# Autodesk Inventor assembly: SG90 - Micro Servo 9g - Tower Pro
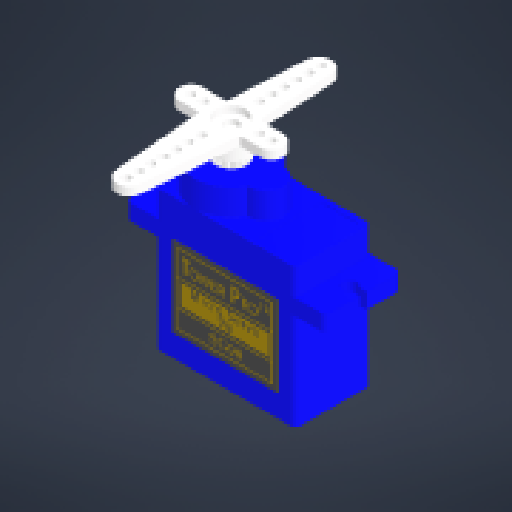
[picture p0: Inventor's stored thumbnail of the model, 512x512]
Saved by Autodesk Inventor 2024 (Build 280153000, 153)
## iProperties
Created: 2019-03-11
Part Number: SG90 - Micro Servo 9g - Tower Pro
Description: STEP AP214
Document SubType Name: Assembly
Designer: Daniel
Sending System: SolidWorks 2018
Preprocessor: SwSTEP 2.0
Title: SG90 - Micro Servo 9g - Tower Pro.STEP
Revision Number: ANY
## Documents named in this file (3)
- C:\Users\Daniel\Desktop\pmik_2024l_jd\mechanical\STEPS\SG90 - Micro Servo 9g - Tower Pro.iam
- C:\Users\Daniel\Desktop\pmik_2024l_jd\mechanical\STEPS\SG90 - Micro Servo 9g - Tower Pro.1_Pea.ipt
- C:\Users\Daniel\Desktop\pmik_2024l_jd\mechanical\STEPS\SG90 - Micro Servo 9g - Tower Pro.4_Pea.ipt
## Components (2 placed, 2 different names)
1. SG90 - Micro Servo 9g - Tower Pro.1_Pea_1 — Cylindrical:1, Angle:1, Mate:1
2. SG90 - Micro Servo 9g - Tower Pro.4_Pea_4 — Cylindrical:1, Angle:1, Mate:1
## Relationships (3: CylindricalJoint 1, Angle 1, Mate 1)
- Cylindrical:1: SG90 - Micro Servo 9g - Tower Pro.1_Pea_1 ↔ SG90 - Micro Servo 9g - Tower Pro.4_Pea_4
- Angle:1 (0 deg): SG90 - Micro Servo 9g - Tower Pro.1_Pea_1 ↔ SG90 - Micro Servo 9g - Tower Pro.4_Pea_4
- Mate:1 (0.5 mm): SG90 - Micro Servo 9g - Tower Pro.1_Pea_1 ↔ SG90 - Micro Servo 9g - Tower Pro.4_Pea_4
